# Autodesk Inventor assembly: Ring Shooter
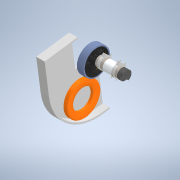
[picture p0: Inventor's stored thumbnail of the model, 180x180]
Saved by Autodesk Inventor 2020 (Build 240168000, 168)
## iProperties
Created: 2020-09-29
Part Number: Ring Shooter
Document SubType Name: Assembly
Designer: jackm
Author: jackm
## Documents named in this file (5)
- D:\FTC8863\2020 Robot\Ring Shooter (one Wheel)\Ring Shooter.iam
- D:\downloads2\am-4300 Ring.ipt
- D:\FTC8863\2019 Robot\Collection\neverest 40 + mounts.iam
- D:\FTC8863\Andymark\am-2648_4inWheel8mmHub.ipt
- D:\FTC8863\2020 Robot\Ring Shooter (one Wheel)\Ring Shooter guide.ipt
## Components (4 placed, 4 different names)
1. am-4300 Ring:1 — Flush:2, Mate:2, Flush:3, Flush:4
2. neverest 40 + mounts:1 [sub-assembly] — Mate:1, Flush:1
3. am-2648_4inWheel8mmHub:1 — Mate:1, Flush:1, Flush:2, Mate:2
4. Ring Shooter guide:1 — Flush:3, Flush:4
## Relationships (6: Flush 4, Mate 2)
- Mate:1: neverest 40 + mounts:1 ↔ am-2648_4inWheel8mmHub:1
- Flush:1: neverest 40 + mounts:1 ↔ am-2648_4inWheel8mmHub:1
- Flush:2: am-4300 Ring:1 ↔ am-2648_4inWheel8mmHub:1
- Mate:2 (114.3 mm): am-4300 Ring:1 ↔ am-2648_4inWheel8mmHub:1
- Flush:3: am-4300 Ring:1 ↔ Ring Shooter guide:1
- Flush:4: am-4300 Ring:1 ↔ Ring Shooter guide:1
